# Autodesk Inventor assembly: Rebreather-HoseAdapter-Assy
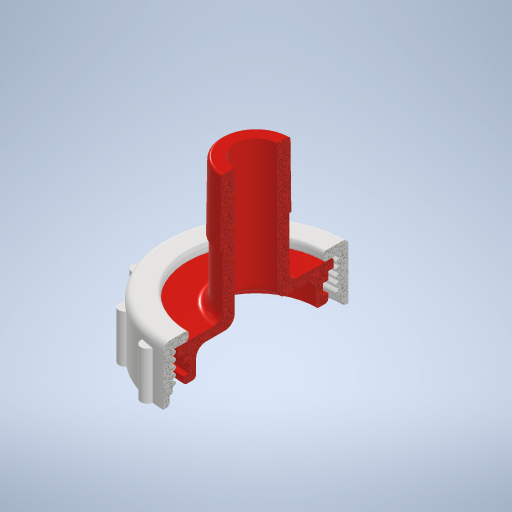
[picture p0: Inventor's stored thumbnail of the model, 512x512]
Saved by Autodesk Inventor 2023 (Build 270158000, 158)
## iProperties
Created: 2022-11-09
Part Number: Rebreather-HoseAdapter-Assy
Document SubType Name: Assembly
Designer: incep
Author: incep
## Documents named in this file (3)
- C:\Users\incep\OneDrive\Desktop\3D Printer Stuff\Rebreather-HoseAdapter-Assy.iam
- C:\Users\incep\OneDrive\Desktop\3D Printer Stuff\Rebreather-HoseRetainer.ipt
- C:\Users\incep\OneDrive\Desktop\3D Printer Stuff\Rebreather-HoseAdapterInsert.ipt
## Components (2 placed, 2 different names)
1. Rebreather-HoseRetainer:1 — Mate:2, Mate:3
2. Rebreather-HoseAdapterInsert:1 — Mate:1, Flush:1, Mate:2, Mate:3
## Relationships (4: Mate 3, Flush 1)
- Mate:1: Rebreather-HoseAdapterInsert:1
- Flush:1: Rebreather-HoseAdapterInsert:1
- Mate:2: Rebreather-HoseRetainer:1 ↔ Rebreather-HoseAdapterInsert:1
- Mate:3: Rebreather-HoseRetainer:1 ↔ Rebreather-HoseAdapterInsert:1
